# Autodesk Inventor assembly: Assembly2
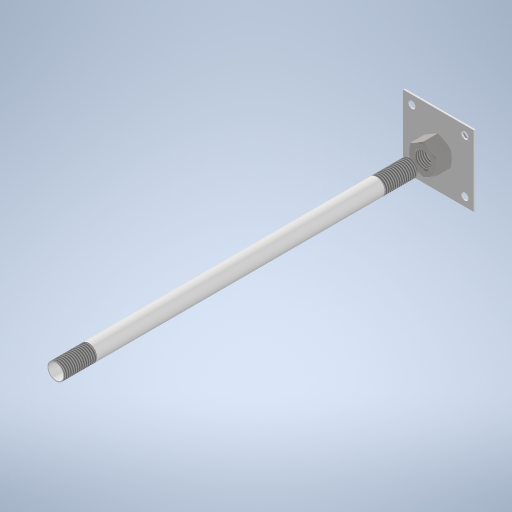
[picture p0: Inventor's stored thumbnail of the model, 512x512]
Saved by Autodesk Inventor 2023 (Build 270158000, 158)
## iProperties
Created: 2022-09-29
Part Number: Assembly2
Document SubType Name: Assembly
Designer: earls
Author: earls
## Documents named in this file (4)
- C:\Users\earls\Documents\stewart-platform\CAD\Smoke generator\Assembly2.iam
- C:\Users\earls\OneDrive\Documents\Inventor\Content Center Files\R2023\en-US\ANSI B 18.2.4.1 M(1)\ANSI B 18.2.4.1 M - M20 x 2.5Style 1.ipt
- C:\Users\earls\Documents\stewart-platform\CAD\Smoke generator\Threaded pipe.ipt
- C:\Users\earls\Documents\stewart-platform\CAD\Smoke generator\plate.ipt
## Components (4 placed, 3 different names)
1. Hex Nut Metric M20 x 2.5:1 — Cylindrical:1, Mate:1, Mate:4
2. Threaded pipe:1 — Cylindrical:1, Mate:2
3. plate:1 — Mate:1, Mate:2, Mate:3
4. Hex Nut Metric M20 x 2.5:2 — Mate:3, Mate:4
## Relationships (5: Mate 4, CylindricalJoint 1)
- Cylindrical:1: Hex Nut Metric M20 x 2.5:1 ↔ Threaded pipe:1
- Mate:1: Hex Nut Metric M20 x 2.5:1 ↔ plate:1
- Mate:2: Threaded pipe:1 ↔ plate:1
- Mate:3: plate:1 ↔ Hex Nut Metric M20 x 2.5:2
- Mate:4: Hex Nut Metric M20 x 2.5:1 ↔ Hex Nut Metric M20 x 2.5:2
